# Autodesk Inventor assembly: nanotwister_reaper
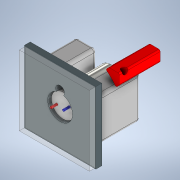
[picture p0: Inventor's stored thumbnail of the model, 180x180]
Saved by Autodesk Inventor 2021 (Build 250183000, 183)
## iProperties
Created: 2022-02-27
Part Number: nanotwister_reaper
Document SubType Name: Assembly
Designer: ermoz
Author: ermoz
## Documents named in this file (6)
- D:\Moje Wyczyny\My_Poor_Projects\nanosumo-nanotwister\mechanics\nanotwister_reaper.iam
- D:\Moje Wyczyny\My_Poor_Projects\nanosumo-nanotwister\mechanics\motor_noname.ipt
- D:\Moje Wyczyny\My_Poor_Projects\nanosumo-nanotwister\mechanics\pb_hole.ipt
- D:\Moje Wyczyny\My_Poor_Projects\nanosumo-nanotwister\mechanics\hot_glue_mashroom.ipt
- D:\Moje Wyczyny\My_Poor_Projects\nanosumo-nanotwister\mechanics\battery_1S_100mAh_no_prot.ipt
- D:\Moje Wyczyny\My_Poor_Projects\nanosumo-nanotwister\mechanics\rotor_core.ipt
## Components (6 placed, 5 different names)
1. motor_noname:1 — Mate:1, Mate:5, Tangent:1, Tangent:2, Mate:8, Flush:4
2. pb_hole:1 — Mate:1, Mate:4, Flush:2, Flush:3, Mate:6, Mate:7, Angle:1, Angle:2
3. hot_glue_mashroom:1 — Mate:4, Flush:2, Flush:3, Mate:5
4. battery_1S_100mAh_no_prot:1 — Mate:6, Tangent:1, Angle:1
5. battery_1S_100mAh_no_prot:2 — Mate:7, Tangent:2, Angle:2
6. rotor_core:1 — Mate:8, Flush:4
## Relationships (13: Mate 6, Flush 3, Tangent 2, Angle 2)
- Mate:1: motor_noname:1 ↔ pb_hole:1
- Mate:4: pb_hole:1 ↔ hot_glue_mashroom:1
- Flush:2 (0.25 mm): pb_hole:1 ↔ hot_glue_mashroom:1
- Flush:3 (0.25 mm): pb_hole:1 ↔ hot_glue_mashroom:1
- Mate:5 (1 mm): motor_noname:1 ↔ hot_glue_mashroom:1
- Mate:6: pb_hole:1 ↔ battery_1S_100mAh_no_prot:1
- Mate:7: pb_hole:1 ↔ battery_1S_100mAh_no_prot:2
- Tangent:1: motor_noname:1 ↔ battery_1S_100mAh_no_prot:1
- Tangent:2: motor_noname:1 ↔ battery_1S_100mAh_no_prot:2
- Angle:1 (0 deg): pb_hole:1 ↔ battery_1S_100mAh_no_prot:1
- Angle:2 (0 deg): pb_hole:1 ↔ battery_1S_100mAh_no_prot:2
- Mate:8: motor_noname:1 ↔ rotor_core:1
- Flush:4 (-0.5 mm): motor_noname:1 ↔ rotor_core:1
